# Autodesk Inventor assembly: shoot
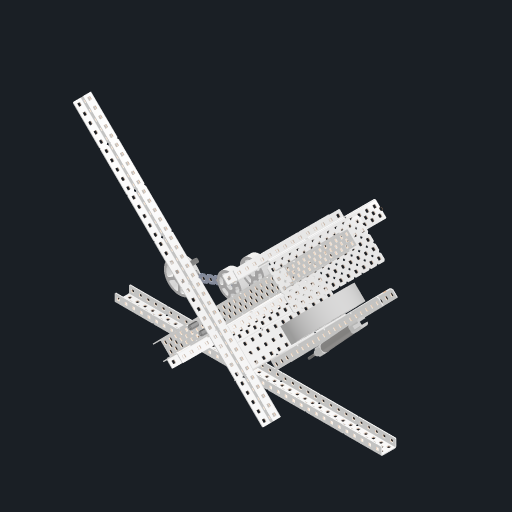
[picture p0: Inventor's stored thumbnail of the model, 512x512]
Saved by Autodesk Inventor 2023 (Build 270158000, 158)
## iProperties
Created: 2023-04-08
Part Number: shoot
Document SubType Name: Assembly
Designer: Windows Macbook
Author: Windows Macbook
## Documents named in this file (17)
- C:\Users\Windows Macbook\Desktop\VRC-SPIN-UP\Inventor\Assembly\Worlds\shoot.iam
- C:\Users\Windows Macbook\Desktop\VRC-SPIN-UP\Inventor\Structure\C Channel\Aluminum 1x2x1\Alu C 1x2x1x35.ipt
- C:\Users\Windows Macbook\Desktop\VRC-SPIN-UP\Inventor\Structure\Standoff\Standoff .50.ipt
- C:\Users\Windows Macbook\Desktop\VRC-SPIN-UP\Inventor\Structure\Standoff.ipt
- C:\Users\Windows Macbook\Desktop\VRC-SPIN-UP\Inventor\Structure\Angle\Aluminum\2x2\Alu Angle 2x2x14.ipt
- C:\Users\Windows Macbook\Desktop\VRC-SPIN-UP\Inventor\Motion\Wheels\Flex Wheels\2.000 Flex Wheel\2.000 30A .500.ipt
- C:\Users\Windows Macbook\Desktop\VRC-SPIN-UP\Inventor\Motion\Wheels\Flex Wheels\2.000 Flex Wheel.ipt
- C:\Users\Windows Macbook\Desktop\VRC-SPIN-UP\Inventor\Motion\Wheels\Flex Wheels\1.625 Flex Wheel\1.625 30A .500.ipt
- C:\Users\Windows Macbook\Desktop\VRC-SPIN-UP\Inventor\Motion\Wheels\Flex Wheels\1.625 Flex Wheel.ipt
- C:\Users\Windows Macbook\Desktop\VRC-SPIN-UP\Inventor\Structure\Plate\Steel\Steel Plate 1x8.ipt
- C:\Users\Windows Macbook\Desktop\VRC-SPIN-UP\Inventor\Structure\C Channel\Aluminum 1x2x1\Alu C 1x2x1x14.ipt
- C:\Users\Windows Macbook\Desktop\VRC-SPIN-UP\Inventor\Structure\C Channel\Aluminum 1x2x1\Alu C 1x2x1x20.ipt
- C:\Users\Windows Macbook\Desktop\VRC-SPIN-UP\Inventor\Structure\C Channel\Aluminum 1x3x1\Alu C 1x3x1x14.ipt
- C:\Users\Windows Macbook\Desktop\VRC-SPIN-UP\Inventor\Motion\Wheels\Flex Wheels\4.000 Flex Wheel\4.000 30A 1.000.ipt
- C:\Users\Windows Macbook\Desktop\VRC-SPIN-UP\Inventor\Motion\Wheels\Flex Wheels\4.000 Flex Wheel.ipt
- C:\Users\Windows Macbook\Desktop\VRC-SPIN-UP\Inventor\Motion\Pneumatics\Double Acting Piston.iam
- C:\Users\Windows Macbook\Desktop\VRC-SPIN-UP\Inventor\Structure\Plate\Aluminum\Alu Plate 5x12.ipt
## Components (20 placed, 12 different names)
1. Alu C 1x2x1x35:1 — Insert:7, Insert:8
2. Alu C 1x2x1x35:2 — Insert:3, Insert:4
3. Standoff .50:1 — Insert:3
4. Standoff .50:2 — Insert:4
5. Alu Angle 2x2x14:1
6. 2.000 30A .500:1
7. 1.625 30A .500:1
8. 1.625 30A .500:2
9. Standoff .50:3 — Insert:8
10. Standoff .50:4 — Insert:7
11. Steel Plate 1x8:1
12. Alu C 1x2x1x14:1
13. Alu C 1x2x1x14:2
14. Alu C 1x3x1x14:1
15. Alu C 1x2x1x20:1
16. 4.000 30A 1.000:1
17. Alu C 1x2x1x35:3
18. Double Acting Piston:1 [sub-assembly]
19. Alu C 1x2x1x14:3
20. Alu Plate 5x12:1
## Relationships (4: Insert 4)
- Insert:3: Alu C 1x2x1x35:2 ↔ Standoff .50:1
- Insert:4: Alu C 1x2x1x35:2 ↔ Standoff .50:2
- Insert:7: Alu C 1x2x1x35:1 ↔ Standoff .50:4
- Insert:8: Alu C 1x2x1x35:1 ↔ Standoff .50:3
